# Autodesk Inventor assembly: set2_to_print_modified
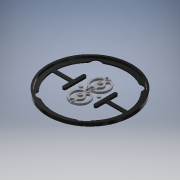
[picture p0: Inventor's stored thumbnail of the model, 180x180]
Saved by Autodesk Inventor 2017 SP1 (Build 210196100, 196)
## iProperties
Created: 2016-07-26
Part Number: set2_to_print_modified
Material: Générique
Document SubType Name: Assembly
Designer: tmonglon
Author: tmonglon
## Documents named in this file (4)
- D:\Inventor\Ahmet\ebug-chassis-june2017\design-jul2017\design - Copie\set2_to_print.iam
- D:\Inventor\Ahmet\mai_2017\modified\bumper_modified2.ipt
- D:\Inventor\Ahmet\29_mai_2017\20170525_ebug_chassis\plug_small_magnet5_holder.ipt
- D:\Inventor\Ahmet\29_mai_2017\20170525_ebug_chassis\small_magnet_holder5.ipt
## Components (5 placed, 3 different names)
1. bumper_modified2:1 — Placage:1, Placage:2, Affleurement:1, Placage:3, Placage:4, Affleurement:6, Affleurement:7, Placage:7, Placage:8, Placage:9, Placage:10
2. plug_small_magnet5_holder:1 — Affleurement:6, Placage:7
3. plug_small_magnet5_holder:2 — Affleurement:7, Placage:8
4. small_magnet_holder5:1 — Affleurement:2, Placage:4, Placage:9
5. small_magnet_holder5:2 — Affleurement:3, Placage:3, Placage:10
## Relationships (13: Mate 8, Flush 5)
- Placage:1 [Mate]: bumper_modified2:1
- Placage:2 [Mate]: bumper_modified2:1
- Affleurement:1 [Flush]: bumper_modified2:1
- Affleurement:2 [Flush]: small_magnet_holder5:1
- Affleurement:3 [Flush]: small_magnet_holder5:2
- Placage:3 [Mate]: bumper_modified2:1 ↔ small_magnet_holder5:2
- Placage:4 [Mate]: bumper_modified2:1 ↔ small_magnet_holder5:1
- Affleurement:6 [Flush]: bumper_modified2:1 ↔ plug_small_magnet5_holder:1
- Affleurement:7 [Flush]: bumper_modified2:1 ↔ plug_small_magnet5_holder:2
- Placage:7 [Mate]: bumper_modified2:1 ↔ plug_small_magnet5_holder:1
- Placage:8 [Mate]: bumper_modified2:1 ↔ plug_small_magnet5_holder:2
- Placage:9 [Mate] (-15 mm): bumper_modified2:1 ↔ small_magnet_holder5:1
- Placage:10 [Mate] (15 mm): bumper_modified2:1 ↔ small_magnet_holder5:2
